# Autodesk Inventor assembly: untitled.brd
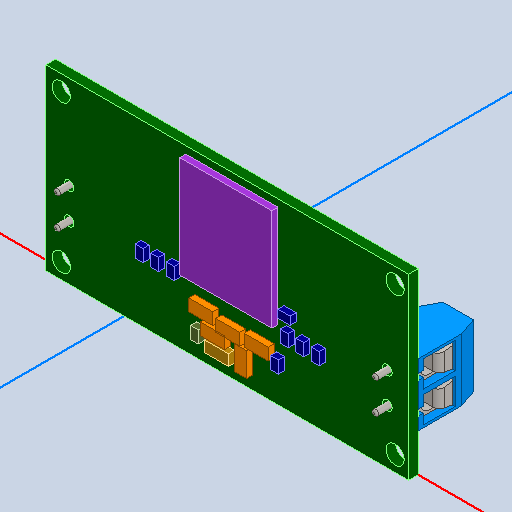
[picture p0: Inventor's stored thumbnail of the model, 512x512]
Saved by Autodesk Inventor 2022 (Build 260153000, 153)
## iProperties
Created: 2022-02-26
Part Number: untitled.brd
Document SubType Name: Assembly
Designer: Petrov Ivan
Author: Petrov Ivan
## Documents named in this file (8)
- D:\IVAN\Ivan_desktop\Kvantorium\Projects\YouBotRobot\electronic\jetson_power_board\untitled.brd.iam
- D:\IVAN\Ivan_desktop\Kvantorium\Projects\YouBotRobot\electronic\jetson_power_board\untitled.brdКонтур.ipt
- D:\IVAN\Ivan_desktop\Kvantorium\Projects\YouBotRobot\electronic\jetson_power_board\C0805K, C0805K_1.ipt
- D:\IVAN\Ivan_desktop\Kvantorium\Projects\YouBotRobot\electronic\jetson_power_board\SOD-123_MINI-SMA, CGRM4004-G_13.ipt
- D:\IVAN\Ivan_desktop\Kvantorium\Projects\YouBotRobot\electronic\jetson_power_board\CHIPLED_0805, CHIPLED_0805_19.ipt
- D:\IVAN\Ivan_desktop\Kvantorium\Projects\YouBotRobot\electronic\jetson_power_board\R0805, R0805_21.ipt
- D:\IVAN\Ivan_desktop\Kvantorium\Projects\YouBotRobot\electronic\jetson_power_board\LMZ13610, LMZ13610_27.ipt
- D:\IVAN\Ivan_desktop\Kvantorium\Projects\YouBotRobot\electronic\jetson_power_board\Terminal Block 2P.ipt
## Components (19 placed, 7 different names)
1. untitled.brdКонтур.ipt:1 — Совмещение:1, Совмещение:2, Угол:1, Совмещение:3, Совмещение:4, Угол:2
2. C0805K, C0805K_1.ipt:1
3. C0805K, C0805K_1.ipt:2
4. C0805K, C0805K_1.ipt:3
5. C0805K, C0805K_1.ipt:4
6. C0805K, C0805K_1.ipt:5
7. C0805K, C0805K_1.ipt:6
8. C0805K, C0805K_1.ipt:7
9. C0805K, C0805K_1.ipt:8
10. SOD-123_MINI-SMA, CGRM4004-G_13.ipt:1
11. CHIPLED_0805, CHIPLED_0805_19.ipt:1
12. R0805, R0805_21.ipt:1
13. R0805, R0805_21.ipt:2
14. R0805, R0805_21.ipt:3
15. R0805, R0805_21.ipt:4
16. R0805, R0805_21.ipt:5
17. LMZ13610, LMZ13610_27.ipt:1
18. Terminal Block 2P.ipt:1 — Совмещение:3, Совмещение:4, Угол:2
19. Terminal Block 2P.ipt:2 — Совмещение:1, Совмещение:2, Угол:1
## Relationships (6: Mate 4, Angle 2)
- Совмещение:1 [Mate]: untitled.brdКонтур.ipt:1 ↔ Terminal Block 2P.ipt:2
- Совмещение:2 [Mate]: untitled.brdКонтур.ipt:1 ↔ Terminal Block 2P.ipt:2
- Угол:1 [Angle] (0 deg): untitled.brdКонтур.ipt:1 ↔ Terminal Block 2P.ipt:2
- Совмещение:3 [Mate]: untitled.brdКонтур.ipt:1 ↔ Terminal Block 2P.ipt:1
- Совмещение:4 [Mate]: untitled.brdКонтур.ipt:1 ↔ Terminal Block 2P.ipt:1
- Угол:2 [Angle] (0 deg): untitled.brdКонтур.ipt:1 ↔ Terminal Block 2P.ipt:1
